# Autodesk Inventor assembly: ChalkBot_MasterAssem
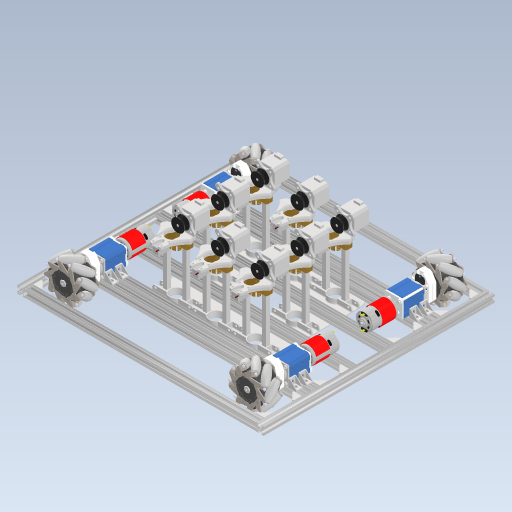
[picture p0: Inventor's stored thumbnail of the model, 512x512]
Saved by Autodesk Inventor 2023 (Build 270158000, 158)
## iProperties
Created: 2022-11-09
Part Number: ChalkBot_MasterAssem
Document SubType Name: Assembly
Designer: Dave
Author: Dave
## Documents named in this file (10)
- C:\Users\Dave\Documents\GrabCAD\Chalk Bot\Chalkbot1.0\ChalkBot_MasterAssem.iam
- C:\Users\Dave\Documents\GrabCAD\Chalk Bot\Chalkbot1.0\Apparatus\V5\8Pc Base Assembly.iam
- C:\Users\Dave\Documents\GrabCAD\Chalk Bot\Chalkbot1.0\Chassis\V1\20x20 Channel.ipt
- C:\Users\Dave\Documents\GrabCAD\Chalk Bot\Chalkbot1.0\Chassis\V1\LeftMecanum-SubAssem01.iam
- C:\Users\Dave\Documents\GrabCAD\Chalk Bot\Chalkbot1.0\Chassis\V1\RightMecanum-SubAssem01.iam
- C:\Users\Dave\Documents\GrabCAD\Chalk Bot\Chalkbot1.0\Chassis\V1\20x20 Channel\20x20 Channel-580.ipt
- C:\Users\Dave\Documents\GrabCAD\Chalk Bot\Chalkbot1.0\Chassis\V1\20x20 90 Gusset.ipt
- C:\Users\Dave\Documents\GrabCAD\Chalk Bot\Chalkbot1.0\Chassis\V1\20x20 90 Gusset_MIR.ipt
- C:\Users\Dave\Documents\GrabCAD\Chalk Bot\Chalkbot1.0\Chassis\V1\20x20 90 Gusset_MIR1.ipt
- C:\Users\Dave\Documents\GrabCAD\Chalk Bot\Chalkbot1.0\Chassis\V1\20x20 90 Gusset_MIR_MIR.ipt
## Components (47 placed, 8 different names)
1. 8Pc Base Assembly:1 [sub-assembly] — Mate:1, Tangent:1, Tangent:2, Flush:18, Mate:3, Tangent:7, Tangent:8, Tangent:9, Tangent:10
2. 20x20 Channel-580:1 — Flush:5, Flush:6, Flush:9, Flush:10, Mate:8, Flush:33, Mate:22, Flush:47, Flush:49
3. 20x20 Channel-580:2 — Flush:6, Flush:7, Flush:8, Flush:9, Flush:27, Flush:28, Mate:4, Mate:5, Mate:6, Symmetry:2, Flush:32
4. 20x20 Channel-580:3 — Flush:7, Flush:8, Mate:1, Flush:15, Flush:16, Flush:18, Mate:12
5. 20x20 Channel-580:4 — Flush:2, Flush:3, Flush:12, Flush:13, Flush:17, Mate:16
6. 20x20 Channel-580:5 — Flush:1, Flush:2, Flush:13, Flush:14, Mate:18
7. 20x20 Channel-580:6 — Flush:1, Flush:14, Flush:29, Symmetry:2, Mate:20
8. 20x20 Channel-580:7 — Flush:3, Flush:4, Flush:11, Flush:12, Flush:16, Flush:17, Mate:15
9. 20x20 Channel-580:8 — Flush:4, Flush:5, Flush:10, Flush:11, Tangent:1, Tangent:2, Flush:15, Mate:11, Flush:48, Flush:50
10. RightMecanum-SubAssem01:2 [sub-assembly]
11. LeftMecanum-SubAssem01:3 [sub-assembly]
12. RightMecanum-SubAssem01:1 [sub-assembly]
13. LeftMecanum-SubAssem01:4 [sub-assembly]
14. 20x20 Channel-580:9 — Flush:27, Flush:28, Mate:4, Flush:29, Flush:30, Flush:31, Mate:7, Mate:9, Flush:34, Mate:10, Mate:13, Flush:35, Mate:14, Mate:17, Mate:19, Mate:21
15. 20x20 Channel-580:10 — Flush:30, Flush:31, Mate:5
16. 20x20 90 Gusset:3 — Flush:34, Mate:10, Mate:11
17. 20x20 90 Gusset:4 — Mate:12, Mate:13, Flush:35, Flush:39
18. 20x20 90 Gusset:6 — Mate:6, Flush:32, Mate:7
19. 20x20 90 Gusset:7 — Mate:8, Mate:9, Flush:33
20. 20x20 90 Gusset_MIR:1 — Flush:36, Flush:37, Mate:16, Mate:17
21. 20x20 90 Gusset_MIR:2 — Flush:36, Flush:39, Mate:14, Mate:15
22. 20x20 90 Gusset_MIR:3 — Flush:38, Mate:20, Mate:21
23. 20x20 90 Gusset_MIR:4 — Flush:37, Flush:38, Mate:18, Mate:19
24. 20x20 90 Gusset_MIR1:1
25. 20x20 90 Gusset_MIR1:2 — Flush:40
26. 20x20 90 Gusset_MIR1:3
27. 20x20 90 Gusset_MIR1:4
28. 20x20 90 Gusset_MIR_MIR:1 — Flush:41, Flush:43
29. 20x20 90 Gusset_MIR_MIR:2 — Flush:40, Flush:41
30. 20x20 90 Gusset_MIR_MIR:3 — Flush:42
31. 20x20 90 Gusset_MIR_MIR:4 — Flush:42, Flush:43
32. 20x20 90 Gusset:8 — Flush:44, Flush:45, Flush:49
33. 20x20 90 Gusset:11 — Flush:44, Flush:50
34. 20x20 90 Gusset:9 — Flush:46, Mate:22, Flush:47
35. 20x20 90 Gusset:10 — Flush:45, Flush:46, Flush:48
36. 20x20 90 Gusset:12
37. 20x20 90 Gusset:13
38. 20x20 90 Gusset:14
39. 20x20 90 Gusset:15
40. 20x20 90 Gusset:16
41. 20x20 90 Gusset:17
42. 20x20 90 Gusset:18
43. 20x20 90 Gusset:19
44. 20x20 90 Gusset:20
45. 20x20 90 Gusset:21
46. 20x20 90 Gusset:22
47. 20x20 90 Gusset:23
## Component patterns: (4 elements, first: 20x20 90 Gusset:8 + 20x20 90 Gusset:11 + 20x20 90 Gusset:9 + 20x20 90 Gusset:10)
## Relationships (88: Flush 50, Mate 26, Tangent 10, Symmetry 2)
- Flush:1: 20x20 Channel-580:5 ↔ 20x20 Channel-580:6
- Flush:2: 20x20 Channel-580:4 ↔ 20x20 Channel-580:5
- Flush:3: 20x20 Channel-580:4 ↔ 20x20 Channel-580:7
- Flush:4: 20x20 Channel-580:7 ↔ 20x20 Channel-580:8
- Flush:5: 20x20 Channel-580:1 ↔ 20x20 Channel-580:8
- Flush:6: 20x20 Channel-580:1 ↔ 20x20 Channel-580:2
- Flush:7: 20x20 Channel-580:2 ↔ 20x20 Channel-580:3
- Flush:8: 20x20 Channel-580:2 ↔ 20x20 Channel-580:3
- Flush:9: 20x20 Channel-580:1 ↔ 20x20 Channel-580:2
- Flush:10: 20x20 Channel-580:1 ↔ 20x20 Channel-580:8
- Flush:11: 20x20 Channel-580:7 ↔ 20x20 Channel-580:8
- Flush:12: 20x20 Channel-580:4 ↔ 20x20 Channel-580:7
- Flush:13: 20x20 Channel-580:4 ↔ 20x20 Channel-580:5
- Flush:14: 20x20 Channel-580:5 ↔ 20x20 Channel-580:6
- Mate:1: 8Pc Base Assembly:1 ↔ 20x20 Channel-580:3
- Tangent:1 (-1.6637 mm): 8Pc Base Assembly:1 ↔ 20x20 Channel-580:8
- Tangent:2 (-1.6637 mm): 8Pc Base Assembly:1 ↔ 20x20 Channel-580:8
- Flush:15 (93 mm): 20x20 Channel-580:3 ↔ 20x20 Channel-580:8
- Flush:16 (93 mm): 20x20 Channel-580:3 ↔ 20x20 Channel-580:7
- Flush:17 (93 mm): 20x20 Channel-580:4 ↔ 20x20 Channel-580:7
- Flush:18 (140 mm): 8Pc Base Assembly:1 ↔ 20x20 Channel-580:3
- [Flush]: RightMecanum-SubAssem01:1 ↔ LeftMecanum-SubAssem01:4
- [Flush]: RightMecanum-SubAssem01:2 ↔ LeftMecanum-SubAssem01:4
- [Flush]: RightMecanum-SubAssem01:2 ↔ LeftMecanum-SubAssem01:3
- [Mate]: 20x20 Channel-580:2 ↔ LeftMecanum-SubAssem01:4
- [Tangent] (1.0795 mm): 20x20 Channel-580:1 ↔ RightMecanum-SubAssem01:1
- [Tangent] (1.0795 mm): 20x20 Channel-580:8 ↔ RightMecanum-SubAssem01:1
- [Tangent] (1.0795 mm): 20x20 Channel-580:5 ↔ LeftMecanum-SubAssem01:3
- [Tangent] (1.331 mm): 20x20 Channel-580:4 ↔ LeftMecanum-SubAssem01:3
- [Flush]: RightMecanum-SubAssem01:2 ↔ LeftMecanum-SubAssem01:3
- [Flush]: LeftMecanum-SubAssem01:3 ↔ RightMecanum-SubAssem01:1
- [Flush]: RightMecanum-SubAssem01:2 ↔ LeftMecanum-SubAssem01:4
- Mate:3: 8Pc Base Assembly:1
- Tangent:7 (-14 mm): 8Pc Base Assembly:1
- Tangent:8 (-14 mm): 8Pc Base Assembly:1
- [Symmetry]: RightMecanum-SubAssem01:1 ↔ LeftMecanum-SubAssem01:4
- [Flush] (462.7118 mm): RightMecanum-SubAssem01:1 ↔ LeftMecanum-SubAssem01:4
- [Flush]: RightMecanum-SubAssem01:1 ↔ LeftMecanum-SubAssem01:4
- Flush:27: 20x20 Channel-580:2 ↔ 20x20 Channel-580:9
- Flush:28: 20x20 Channel-580:2 ↔ 20x20 Channel-580:9
- Mate:4: 20x20 Channel-580:2 ↔ 20x20 Channel-580:9
- Flush:29: 20x20 Channel-580:6 ↔ 20x20 Channel-580:9
- Flush:30: 20x20 Channel-580:9 ↔ 20x20 Channel-580:10
- Flush:31: 20x20 Channel-580:9 ↔ 20x20 Channel-580:10
- Mate:5: 20x20 Channel-580:2 ↔ 20x20 Channel-580:10
- Mate:6: 20x20 Channel-580:2 ↔ 20x20 90 Gusset:6
- Tangent:9 (-14 mm): 8Pc Base Assembly:1
- Tangent:10 (-14 mm): 8Pc Base Assembly:1
- Symmetry:2: 20x20 Channel-580:2 ↔ 20x20 Channel-580:6
- Flush:32: 20x20 Channel-580:2 ↔ 20x20 90 Gusset:6
- Mate:7: 20x20 Channel-580:9 ↔ 20x20 90 Gusset:6
- Mate:8: 20x20 Channel-580:1 ↔ 20x20 90 Gusset:7
- Mate:9: 20x20 Channel-580:9 ↔ 20x20 90 Gusset:7
- Flush:33: 20x20 Channel-580:1 ↔ 20x20 90 Gusset:7
- Flush:34: 20x20 Channel-580:9 ↔ 20x20 90 Gusset:3
- Mate:10: 20x20 Channel-580:9 ↔ 20x20 90 Gusset:3
- Mate:11: 20x20 Channel-580:8 ↔ 20x20 90 Gusset:3
- Mate:12: 20x20 Channel-580:3 ↔ 20x20 90 Gusset:4
- Mate:13: 20x20 Channel-580:9 ↔ 20x20 90 Gusset:4
- Flush:35: 20x20 Channel-580:9 ↔ 20x20 90 Gusset:4
- Flush:36: 20x20 90 Gusset_MIR:1 ↔ 20x20 90 Gusset_MIR:2
- Flush:37: 20x20 90 Gusset_MIR:1 ↔ 20x20 90 Gusset_MIR:4
- Flush:38: 20x20 90 Gusset_MIR:3 ↔ 20x20 90 Gusset_MIR:4
- Flush:39: 20x20 90 Gusset:4 ↔ 20x20 90 Gusset_MIR:2
- Mate:14: 20x20 Channel-580:9 ↔ 20x20 90 Gusset_MIR:2
- Mate:15: 20x20 Channel-580:7 ↔ 20x20 90 Gusset_MIR:2
- Mate:16: 20x20 Channel-580:4 ↔ 20x20 90 Gusset_MIR:1
- Mate:17: 20x20 Channel-580:9 ↔ 20x20 90 Gusset_MIR:1
- Mate:18: 20x20 Channel-580:5 ↔ 20x20 90 Gusset_MIR:4
- Mate:19: 20x20 Channel-580:9 ↔ 20x20 90 Gusset_MIR:4
- Mate:20: 20x20 Channel-580:6 ↔ 20x20 90 Gusset_MIR:3
- Mate:21: 20x20 Channel-580:9 ↔ 20x20 90 Gusset_MIR:3
- Flush:40: 20x20 90 Gusset_MIR1:2 ↔ 20x20 90 Gusset_MIR_MIR:2
- Flush:41: 20x20 90 Gusset_MIR_MIR:1 ↔ 20x20 90 Gusset_MIR_MIR:2
- Flush:42: 20x20 90 Gusset_MIR_MIR:3 ↔ 20x20 90 Gusset_MIR_MIR:4
- Flush:43: 20x20 90 Gusset_MIR_MIR:1 ↔ 20x20 90 Gusset_MIR_MIR:4
- Flush:44: 20x20 90 Gusset:8 ↔ 20x20 90 Gusset:11
- Flush:45: 20x20 90 Gusset:8 ↔ 20x20 90 Gusset:10
- Flush:46: 20x20 90 Gusset:9 ↔ 20x20 90 Gusset:10
- Mate:22: 20x20 Channel-580:1 ↔ 20x20 90 Gusset:9
- [Mate]: RightMecanum-SubAssem01:1 ↔ 20x20 90 Gusset:9
- Flush:47: 20x20 Channel-580:1 ↔ 20x20 90 Gusset:9
- [Mate]: RightMecanum-SubAssem01:1 ↔ 20x20 90 Gusset:10
- Flush:48: 20x20 Channel-580:8 ↔ 20x20 90 Gusset:10
- [Mate]: RightMecanum-SubAssem01:1 ↔ 20x20 90 Gusset:8
- Flush:49: 20x20 Channel-580:1 ↔ 20x20 90 Gusset:8
- [Mate]: RightMecanum-SubAssem01:1 ↔ 20x20 90 Gusset:11
- Flush:50: 20x20 Channel-580:8 ↔ 20x20 90 Gusset:11
